# Autodesk Inventor assembly: motor_wheel_2
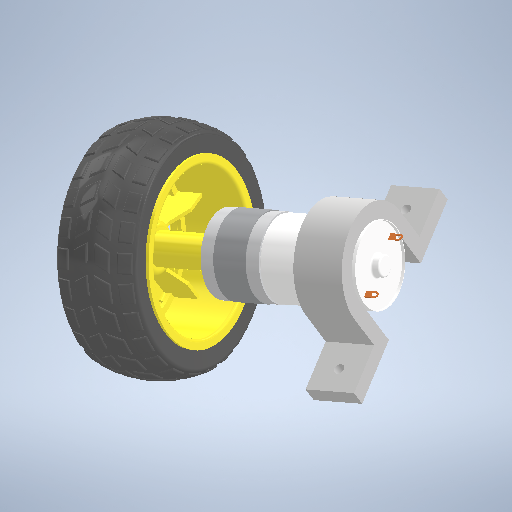
[picture p0: Inventor's stored thumbnail of the model, 512x512]
Saved by Autodesk Inventor 2025.3 (Build 293356030, 356C)
## iProperties
Created: 2026-06-28
Part Number: motor_wheel_2
Document SubType Name: Assembly
Designer: user
Author: user
## Documents named in this file (4)
- C:\Docs\shcool\dojo\Design_3\Smaller\motor_wheel_3.iam
- C:\Docs\shcool\dojo\Design_3\motor_wheel\Geared_motor.ipt
- C:\Docs\shcool\dojo\Design_3\Smaller\imports\Wheel.ipt
- C:\Docs\shcool\dojo\Design_3\Smaller\U_BRACKET_2.ipt
## Components (3 placed, 3 different names)
1. Geared_motor:1 — Insert:1, Insert:2
2. U_BRACKET_2:1 — Insert:1
3. Wheel:1 — Insert:2
## Relationships (2: Insert 2)
- Insert:1: Geared_motor:1 ↔ U_BRACKET_2:1
- Insert:2: Geared_motor:1 ↔ Wheel:1
